# Autodesk Inventor assembly: Claw Assembly
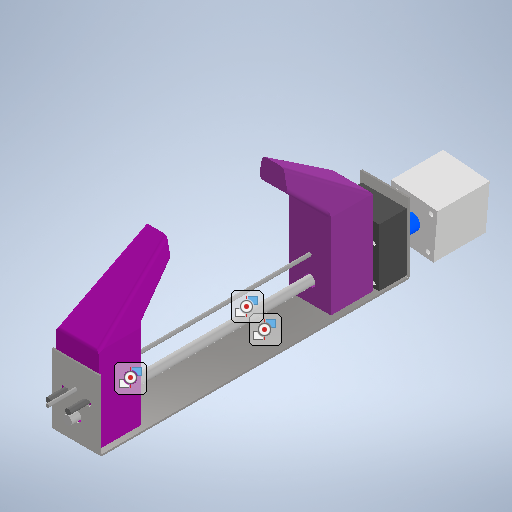
[picture p0: Inventor's stored thumbnail of the model, 512x512]
Saved by Autodesk Inventor 2025.1 (Build 291241020, 241B)
## iProperties
Created: 2025-01-21
Part Number: Claw Assembly
Document SubType Name: Assembly
Designer: Sven
Author: Sven
## Documents named in this file (10)
- C:\Users\aidan\Documents\BehrendURCMechanical\CAD\Arm\Hamburger\BRC Robotic CLaw\Claw Assembly.iam
- C:\Users\aidan\Documents\BehrendURCMechanical\CAD\Arm\Hamburger\BRC Robotic CLaw\Moving Gripper.ipt
- C:\Users\aidan\Documents\BehrendURCMechanical\CAD\Arm\Hamburger\BRC Robotic CLaw\Stationary Gripper.ipt
- C:\Users\aidan\Documents\BehrendURCMechanical\CAD\Arm\Hamburger\BRC Robotic CLaw\Lead Screw.ipt
- C:\Users\aidan\Documents\BehrendURCMechanical\CAD\Arm\Hamburger\BRC Robotic CLaw\#10 2in.ipt
- C:\Users\aidan\Documents\BehrendURCMechanical\CAD\Arm\Hamburger\BRC Robotic CLaw\Support Bar.ipt
- C:\Users\aidan\Documents\BehrendURCMechanical\CAD\Arm\Hamburger\BRC Robotic CLaw\Motor Brace.ipt
- C:\Users\aidan\Documents\BehrendURCMechanical\CAD\Arm\Hamburger\BRC Robotic CLaw\Couple.ipt
- C:\Users\aidan\Documents\BehrendURCMechanical\CAD\Arm\Hamburger\BRC Robotic CLaw\NEMA 17 Completely Correct.ipt
- C:\Users\aidan\Documents\BehrendURCMechanical\CAD\Arm\Hamburger\BRC Robotic CLaw\Bracket (Sheet Metal).ipt
## Components (10 placed, 9 different names)
1. Bracket (Sheet Metal):1 — Mate:3, Mate:4, Mate:15, Mate:28, Mate:30
2. Moving Gripper:1 — Mate:6, Mate:14, Mate:26
3. Stationary Gripper:1 — Mate:4, Mate:7, Mate:8, Mate:9, Mate:10, Mate:11, Mate:14, Mate:30
4. Lead Screw:1 — Mate:3, Mate:6, Mate:7, Mate:20, Mate:21, Mate:25
5. #10 2in:1 — Mate:8, Mate:9
6. #10 2in:2 — Mate:10, Mate:11
7. Support Bar:1 — Mate:15, Mate:26, Mate:27
8. Motor Brace:1 — Mate:27, Mate:28
9. Couple:1 — Mate:20, Mate:21, Mate:24
10. NEMA 17 Completely Correct:1 — Mate:24, Mate:25
## Relationships (18: Mate 18)
- Mate:3: Bracket (Sheet Metal):1 ↔ Lead Screw:1
- Mate:4: Bracket (Sheet Metal):1 ↔ Stationary Gripper:1
- Mate:6: Moving Gripper:1 ↔ Lead Screw:1
- Mate:7: Stationary Gripper:1 ↔ Lead Screw:1
- Mate:8: Stationary Gripper:1 ↔ #10 2in:1
- Mate:9: Stationary Gripper:1 ↔ #10 2in:1
- Mate:10: Stationary Gripper:1 ↔ #10 2in:2
- Mate:11: Stationary Gripper:1 ↔ #10 2in:2
- Mate:14: Moving Gripper:1 ↔ Stationary Gripper:1
- Mate:15: Bracket (Sheet Metal):1 ↔ Support Bar:1
- Mate:20: Lead Screw:1 ↔ Couple:1
- Mate:21: Lead Screw:1 ↔ Couple:1
- Mate:24: Couple:1 ↔ NEMA 17 Completely Correct:1
- Mate:25: Lead Screw:1 ↔ NEMA 17 Completely Correct:1
- Mate:26: Moving Gripper:1 ↔ Support Bar:1
- Mate:27: Support Bar:1 ↔ Motor Brace:1
- Mate:28: Bracket (Sheet Metal):1 ↔ Motor Brace:1
- Mate:30: Bracket (Sheet Metal):1 ↔ Stationary Gripper:1
